# Autodesk Inventor assembly: FrontWheelFrameNew
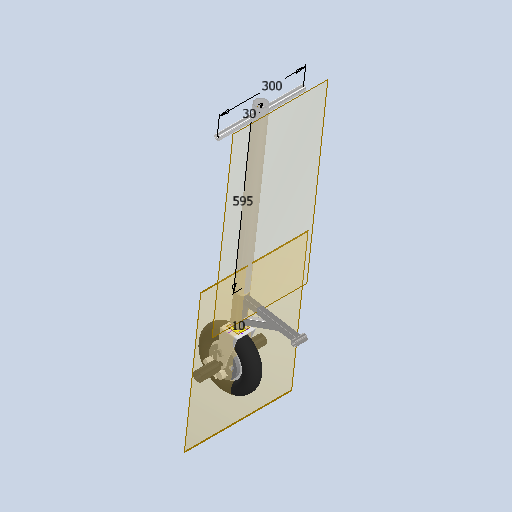
[picture p0: Inventor's stored thumbnail of the model, 512x512]
Saved by Autodesk Inventor 2022.2 (Build 262287000, 287)
## iProperties
Created: 2022-04-06
Part Number: FrontWheelFrameNew
Document SubType Name: Assembly
Designer: Finn Oriwohl
Mass: 2964.03 g
Surface Area: 4560.09 cm^2
Volume: 1772.52 cm^3
Density: 1.67221 g/cm^3
_SolveAssemblyDoc: Frame Generator Solve Assembly
_Version: 25.0.0
Author: Finn Oriwohl
## Documents named in this file (4)
- H:\inventor ting\Mekatronik beercart git\Beercart CAD\Workspaces\Workspace\beercart assembly - mekatronik\Frame\FrontWheelFrameNew.iam
- H:\inventor ting\Mekatronik beercart git\Beercart CAD\Workspaces\Workspace\FrontWheelAssembly.iam
- H:\inventor ting\Mekatronik beercart git\Beercart CAD\Workspaces\Workspace\beercart assembly - mekatronik\Frame\FrontWheelFrameNew\Frame\Frame 1649861603730.iam
- H:\inventor ting\Mekatronik beercart git\Beercart CAD\Workspaces\Workspace\FrontWheelHandle.ipt
## Components (3 placed, 3 different names)
1. FrontWheelAssembly:1 [sub-assembly] — Rigid:1, Insert:1
2. FrontWheelMount Frame 1649861603730:1 [sub-assembly] — Insert:1
3. FrontWheelHandle:1 — Rigid:1
## Relationships (2: WeldJoint 1, Insert 1)
- Rigid:1 [WeldJoint]: FrontWheelAssembly:1 ↔ FrontWheelHandle:1
- Insert:1 (-18 mm): FrontWheelAssembly:1 ↔ FrontWheelMount Frame 1649861603730:1
